# Autodesk Inventor assembly: Assembly (w filler)
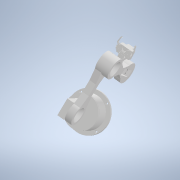
[picture p0: Inventor's stored thumbnail of the model, 180x180]
Saved by Autodesk Inventor 2022 (Build 260153000, 153)
## iProperties
Created: 2022-02-25
Part Number: Assembly (w filler)
Document SubType Name: Assembly
Designer: Alexa
Author: Alexa
## Documents named in this file (9)
- C:\Users\Alexa\Documents\4TH YEAR\ROBOTICS PARTS\Final parts\Assembly (w filler).iam
- C:\Users\Alexa\Documents\4TH YEAR\ROBOTICS PARTS\Final parts\NBase Part.ipt
- C:\Users\Alexa\Documents\4TH YEAR\ROBOTICS PARTS\Final parts\NBase top.ipt
- C:\Users\Alexa\Documents\4TH YEAR\ROBOTICS PARTS\Final parts\1stArm.ipt
- C:\Users\Alexa\Documents\4TH YEAR\ROBOTICS PARTS\Final parts\2ndArm.ipt
- C:\Users\Alexa\Documents\4TH YEAR\ROBOTICS PARTS\Final parts\EndConnector.ipt
- C:\Users\Alexa\Documents\4TH YEAR\ROBOTICS PARTS\Final parts\New Gear.ipt
- C:\Users\Alexa\Documents\4TH YEAR\ROBOTICS PARTS\Final parts\filler.ipt
- C:\Users\Alexa\Documents\4TH YEAR\ROBOTICS PARTS\Final parts\Solo (SG) Gear.ipt
## Components (9 placed, 8 different names)
1. NBase Part:1 — Rotational:1
2. NBase top:1 — Rotational:1, Rotational:2
3. 1stArm:1 — Rotational:2, Rotational:3
4. 2ndArm:1 — Rotational:3, Rotational:4
5. EndConnector:1 — Rotational:4, Rotational:5, Rotational:6, Rotational:7
6. New Gear:1 — Rotational:7
7. New Gear:2 — Rotational:6
8. filler:1 — Rotational:5, Rotational:8
9. Solo (SG) Gear:1 — Rotational:8
## Relationships (8: RevoluteJoint 8)
- Rotational:1 [RevoluteJoint]: NBase Part:1 ↔ NBase top:1
- Rotational:2 [RevoluteJoint]: NBase top:1 ↔ 1stArm:1
- Rotational:3 [RevoluteJoint]: 1stArm:1 ↔ 2ndArm:1
- Rotational:4 [RevoluteJoint]: 2ndArm:1 ↔ EndConnector:1
- Rotational:5 [RevoluteJoint]: EndConnector:1 ↔ filler:1
- Rotational:6 [RevoluteJoint]: EndConnector:1 ↔ New Gear:2
- Rotational:7 [RevoluteJoint]: EndConnector:1 ↔ New Gear:1
- Rotational:8 [RevoluteJoint]: filler:1 ↔ Solo (SG) Gear:1
